# Autodesk Inventor assembly: Welle_V3
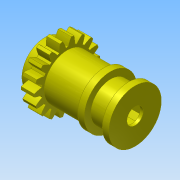
[picture p0: Inventor's stored thumbnail of the model, 180x180]
Saved by Autodesk Inventor 2015 (Build 190159000, 159)
## iProperties
Created: 2015-09-01
Part Number: Welle_V3
Document SubType Name: Assembly
Designer: Johann
Mass: 3.15638 g
Surface Area: 34.0021 cm^2
Volume: 2.97772 cm^3
Density: 1.06 g/cm^3
Author: Johann
## Documents named in this file (3)
- C:\Users\Johann\Documents\Uni\Bachelorarbeit\Inventor\Welle_V4.iam
- C:\Users\Johann\Documents\Uni\Bachelorarbeit\Inventor\Welle_V3\Konstruktions-Assistent\Welle1.iam
- C:\Users\Johann\Documents\Uni\Bachelorarbeit\Inventor\Zahnrad.iam
## Components (2 placed, 2 different names)
1. Welle:1 [sub-assembly] — Fluchtend:1, Fluchtend:2, Fluchtend:3, Passend:1, Passend:2
2. Zahnrad:1 [sub-assembly] — Passend:1, Passend:2
## Relationships (5: Flush 3, Mate 2)
- Fluchtend:1 [Flush]: Welle:1
- Fluchtend:2 [Flush]: Welle:1
- Fluchtend:3 [Flush]: Welle:1
- Passend:1 [Mate]: Welle:1 ↔ Zahnrad:1
- Passend:2 [Mate]: Welle:1 ↔ Zahnrad:1
